# Autodesk Inventor assembly: vertical_stabilizer
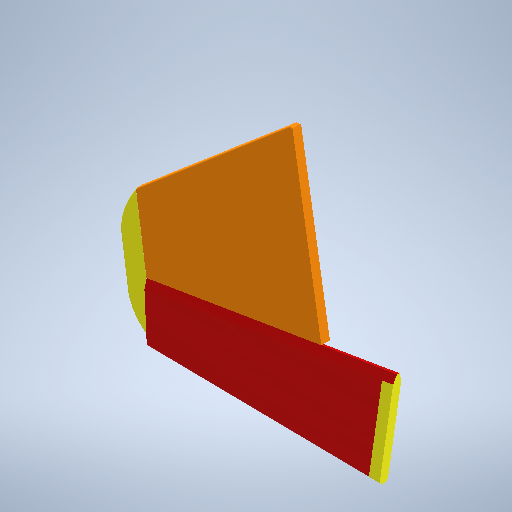
[picture p0: Inventor's stored thumbnail of the model, 512x512]
Saved by Autodesk Inventor 2025.3 (Build 293356000, 356)
## iProperties
Created: 2025-07-09
Part Number: vertical_stabilizer
Document SubType Name: Assembly
Designer: steve
Author: steve
## Documents named in this file (3)
- C:\Users\steve\OneDrive\Documentos\Avion\MODELOS NUEVOS\vertical_stabilizer.iam
- C:\Users\steve\OneDrive\Documentos\Avion\Part13.ipt
- C:\Users\steve\OneDrive\Documentos\Avion\Part14.ipt
## Components (2 placed, 2 different names)
1. Part13:1 — Rotational:1
2. Part14:1 — Rotational:1
## Relationships (1: RevoluteJoint 1)
- Rotational:1 [RevoluteJoint] (22 mm): Part13:1 ↔ Part14:1
## Named parameters: Finish1_Area = 209.692, Finish2_Area = 24.0171, Finish3_Area = 159.152, Finish4_Area = 14.1577
note: some values were not read from the file. Shown as the stored number, unit unknown: "Finish1_Area", "Finish2_Area", "Finish3_Area", "Finish4_Area".
